# Autodesk Inventor assembly: DelrinWheel
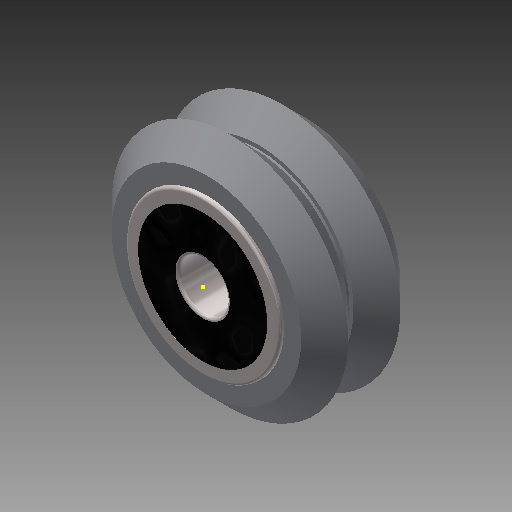
[picture p0: Inventor's stored thumbnail of the model, 512x512]
Saved by Autodesk Inventor 2017 (Build 210142000, 142)
## iProperties
Created: 2016-07-20
Part Number: DelrinWheel
Document SubType Name: Assembly
Designer: User
Author: User
## Documents named in this file (6)
- C:\All INVENTOR\SL-Inventor\SL-Beast 3D Printer\DelrinWheel.iam
- Delrin Wheel.iam
- C:\All INVENTOR\SL-Inventor\SL-Beast 3D Printer\dELRIN.ipt
- C:\All INVENTOR\SL-Inventor\SL-Beast 3D Printer\SKF 625.ipt
- C:\All INVENTOR\SL-Inventor\SL-Beast 3D Printer\SKF 625_CPY.ipt
- C:\All INVENTOR\SL-Inventor\SL-Beast 3D Printer\DelrinShim.ipt
## Components (4 placed, 4 different names)
1. dELRIN:1 — Mate:2, Mate:4, Mate:7, Mate:8
2. SKF 625:1 — Mate:2, Flush:1, Mate:8
3. SKF 625_CPY:1 — Mate:4, Mate:7
4. DelrinShim:1 — Flush:1
## Relationships (5: Mate 4, Flush 1)
- Mate:2: dELRIN:1 ↔ SKF 625:1
- Mate:4: dELRIN:1 ↔ SKF 625_CPY:1
- Flush:1: SKF 625:1 ↔ DelrinShim:1
- Mate:7: dELRIN:1 ↔ SKF 625_CPY:1
- Mate:8: dELRIN:1 ↔ SKF 625:1
